# Autodesk Inventor assembly: Camera Side Panel Assembly
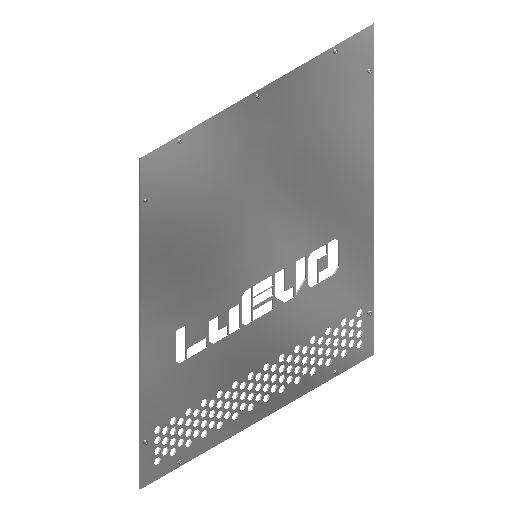
[picture p0: Inventor's stored thumbnail of the model, 512x512]
Saved by Autodesk Inventor 2023.2 (Build 272271000, 271)
## iProperties
Created: 2023-02-06
Part Number: Camera Side Panel Assembly
Document SubType Name: Assembly
Designer: remop
Author: remop
## Documents named in this file (3)
- C:\Users\remop\OneDrive\Documents\Inventor\3D Printers\LuEVO\Mk5_FullKinematic\Camera Side Panel Assembly.iam
- C:\Users\remop\OneDrive\Documents\Inventor\3D Printers\LuEVO\Mk5_FullKinematic\Camera Side Panel.ipt
- C:\Users\remop\OneDrive\Documents\Inventor\Content Center Files\R2023\en-US\AS 1420\AS 1420 - 1973 - M3 x 6.ipt
## Components (10 placed, 2 different names)
1. Camera Side Panel:1 — Insert:1, Insert:2, Insert:3, Insert:4, Insert:5, Insert:6, Insert:7, Insert:8, Insert:9
2. AS 1420 - Metric M3 x 6:1 — Insert:1
3. AS 1420 - Metric M3 x 6:2 — Insert:2
4. AS 1420 - Metric M3 x 6:3 — Insert:3
5. AS 1420 - Metric M3 x 6:4 — Insert:4
6. AS 1420 - Metric M3 x 6:5 — Insert:5
7. AS 1420 - Metric M3 x 6:6 — Insert:6
8. AS 1420 - Metric M3 x 6:7 — Insert:7
9. AS 1420 - Metric M3 x 6:8 — Insert:8
10. AS 1420 - Metric M3 x 6:9 — Insert:9
## Relationships (9: Insert 9)
- Insert:1: Camera Side Panel:1 ↔ AS 1420 - Metric M3 x 6:1
- Insert:2: Camera Side Panel:1 ↔ AS 1420 - Metric M3 x 6:2
- Insert:3: Camera Side Panel:1 ↔ AS 1420 - Metric M3 x 6:3
- Insert:4: Camera Side Panel:1 ↔ AS 1420 - Metric M3 x 6:4
- Insert:5: Camera Side Panel:1 ↔ AS 1420 - Metric M3 x 6:5
- Insert:6: Camera Side Panel:1 ↔ AS 1420 - Metric M3 x 6:6
- Insert:7: Camera Side Panel:1 ↔ AS 1420 - Metric M3 x 6:7
- Insert:8: Camera Side Panel:1 ↔ AS 1420 - Metric M3 x 6:8
- Insert:9: Camera Side Panel:1 ↔ AS 1420 - Metric M3 x 6:9
